# Autodesk Inventor assembly: talp
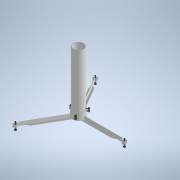
[picture p0: Inventor's stored thumbnail of the model, 180x180]
Saved by Autodesk Inventor 2021.4 (Build 254397000, 397)
## iProperties
Created: 2023-12-02
Part Number: talp
Document SubType Name: Assembly
Designer: vtoth
Author: vtoth
## Documents named in this file (5)
- C:\Users\vtoth\OneDrive - Budapesti Műszaki és Gazdaságtudományi Egyetem\5_felev\CAD\hf2_v2\talp.iam
- C:\Users\vtoth\OneDrive - Budapesti Műszaki és Gazdaságtudományi Egyetem\5_felev\CAD\hf2_v2\haromlab.ipt
- C:\Users\vtoth\OneDrive - Budapesti Műszaki és Gazdaságtudományi Egyetem\5_felev\CAD\hf2_v2\cso.ipt
- C:\Users\vtoth\OneDrive - Budapesti Műszaki és Gazdaságtudományi Egyetem\5_felev\CAD\hf2_v2\ContentCenter\en-US\ISO 4018\ISO 4018 - M8 x 16.ipt
- C:\Users\vtoth\OneDrive - Budapesti Műszaki és Gazdaságtudományi Egyetem\5_felev\CAD\hf2_v2\ContentCenter\en-US\ISO 4018\ISO 4018 - M8 x 50.ipt
## Components (11 placed, 4 different names)
1. haromlab:1 — Mate:1, Mate:2, Flush:1, Mate:3, Mate:4, Mate:5, Flush:7, Flush:2
2. cso:1 — Mate:1, Mate:2, Flush:1, Tangent:1, Tangent:2
3. ISO 4018 M8 x 16:1 — Mate:3, Tangent:1
4. ISO 4018 M8 x 16:2 — Mate:4, Tangent:2
5. ISO 4018 M8 x 50:1 — Mate:5, Flush:7, Flush:2
6. ISO 4018 M8 x 16:3
7. ISO 4018 M8 x 16:4
8. ISO 4018 M8 x 50:2
9. ISO 4018 M8 x 16:5
10. ISO 4018 M8 x 16:6
11. ISO 4018 M8 x 50:3
## Component patterns: (3 elements, first: ISO 4018 M8 x 16:1 + ISO 4018 M8 x 16:2 + ISO 4018 M8 x 50:1)
## Relationships (10: Mate 5, Flush 3, Tangent 2)
- Mate:1: haromlab:1 ↔ cso:1
- Mate:2: haromlab:1 ↔ cso:1
- Flush:1: haromlab:1 ↔ cso:1
- Mate:3: haromlab:1 ↔ ISO 4018 M8 x 16:1
- Tangent:1: cso:1 ↔ ISO 4018 M8 x 16:1
- Mate:4: haromlab:1 ↔ ISO 4018 M8 x 16:2
- Tangent:2: cso:1 ↔ ISO 4018 M8 x 16:2
- Mate:5: haromlab:1 ↔ ISO 4018 M8 x 50:1
- Flush:7 (25 mm): haromlab:1 ↔ ISO 4018 M8 x 50:1
- Flush:2 (25 mm): haromlab:1 ↔ ISO 4018 M8 x 50:1
